# Autodesk Inventor assembly: 4mm_ABD_set
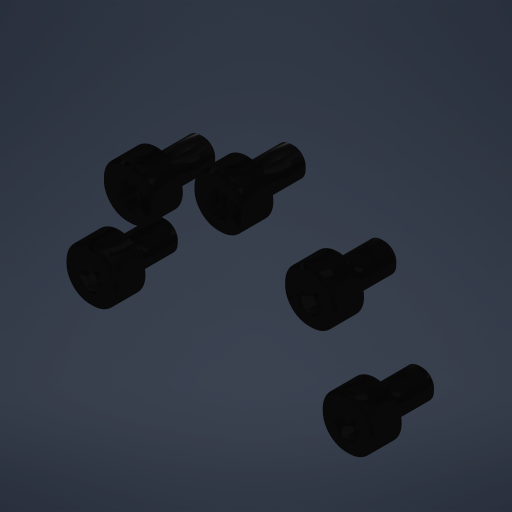
[picture p0: Inventor's stored thumbnail of the model, 512x512]
Saved by Autodesk Inventor 2024 (Build 280153000, 153)
## iProperties
Created: 2024-06-23
Part Number: 4mm_ABD_set
Document SubType Name: Assembly
Designer: ASUS
Author: ASUS
## Documents named in this file (2)
- C:\Users\ASUS\Desktop\2024_Robit_Hardware\ROBOCUP_2024_eindhoven\부품\Bolt_Washer_Nut\4mm_ABD_set.iam
- C:\Users\ASUS\Desktop\2024_Robit_Hardware\ROBOCUP_2024_eindhoven\부품\Bolt_Washer_Nut\CSH-ST-M2_5-4_203.ipt
## Components (5 placed, 1 different names)
1. CSH-ST-M2_5-4_203:1
2. CSH-ST-M2_5-4_203:2
3. CSH-ST-M2_5-4_203:4
4. CSH-ST-M2_5-4_203:5
5. CSH-ST-M2_5-4_203:8
## Relationships (1: Flush 1)
- [Flush]: CSH-ST-M2_5-4_203:1 ↔ CSH-ST-M2_5-4_203:8
